# Autodesk Inventor assembly: 4bar
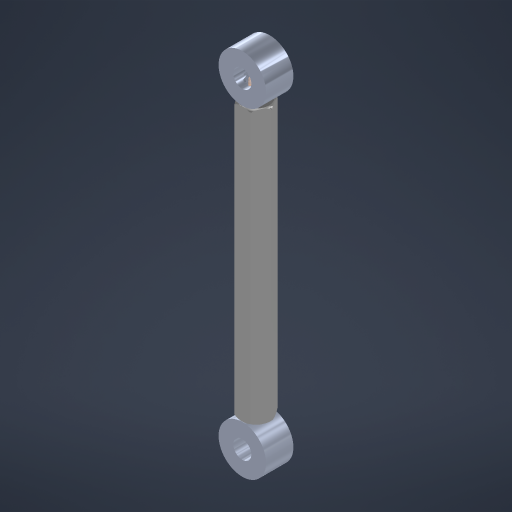
[picture p0: Inventor's stored thumbnail of the model, 512x512]
Saved by Autodesk Inventor 2024 (Build 280153000, 153)
## iProperties
Created: 2023-10-23
Part Number: 4bar
Document SubType Name: Assembly
Designer: macbook
Author: macbook
## Documents named in this file (4)
- \\Mac\Home\Desktop\code\1599V-VRC\Cad\Assembly\v2\4bar.iam
- \\Mac\Home\Desktop\code\1599V-VRC\Cad\Structure\Standoff\Standoff 2.50.ipt
- \\Mac\Home\Desktop\code\1599V-VRC\Cad\Structure\Standoff.ipt
- \\Mac\Home\Desktop\code\1599V-VRC\Cad\Motion\Reference Files\Shaft Collar Metal.ipt
## Components (3 placed, 2 different names)
1. Standoff 2.50:1 — Insert:1, Insert:2
2. Shaft Collar Metal:1 — Insert:1
3. Shaft Collar Metal:2 — Insert:2
## Relationships (2: Insert 2)
- Insert:1: Standoff 2.50:1 ↔ Shaft Collar Metal:1
- Insert:2: Standoff 2.50:1 ↔ Shaft Collar Metal:2
